# Autodesk Inventor assembly: Inverted_pendulum
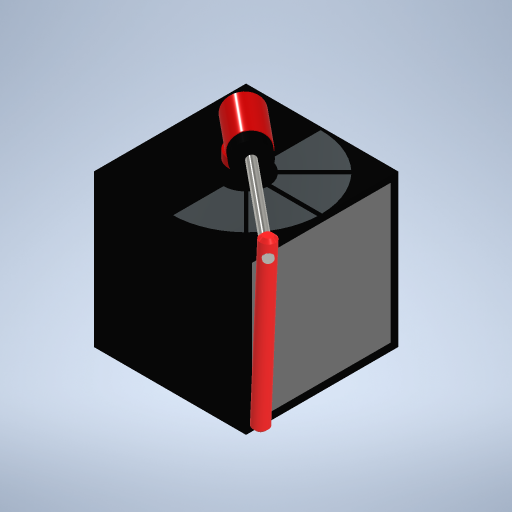
[picture p0: Inventor's stored thumbnail of the model, 512x512]
Saved by Autodesk Inventor 2024 (Build 280153000, 153)
## iProperties
Created: 2024-09-26
Part Number: Inverted_pendulum
Document SubType Name: Assembly
Designer: skcre
Author: skcre
## Documents named in this file (4)
- C:\Users\skcre\Desktop\Qservo\cad\Inverted_pendulum.iam
- C:\Users\skcre\Desktop\Qservo\cad\stepper_box.ipt
- C:\Users\skcre\Desktop\Qservo\cad\encoder.ipt
- C:\Users\skcre\Desktop\Qservo\cad\pendulum.ipt
## Components (3 placed, 3 different names)
1. stepper_box:1 — Mate:1, Mate:2
2. encoder:1 — Mate:1, Mate:2, Mate:3, Mate:4
3. pendulum:1 — Mate:3, Mate:4
## Relationships (4: Mate 4)
- Mate:1: stepper_box:1 ↔ encoder:1
- Mate:2: stepper_box:1 ↔ encoder:1
- Mate:3: encoder:1 ↔ pendulum:1
- Mate:4 (-5 mm): encoder:1 ↔ pendulum:1
